# Autodesk Inventor assembly: AssemblyV1
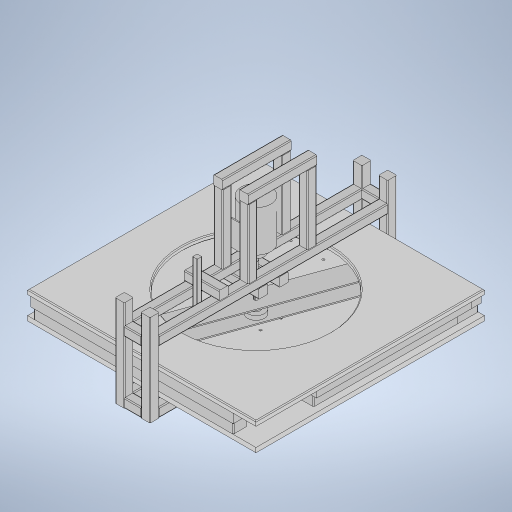
[picture p0: Inventor's stored thumbnail of the model, 512x512]
Saved by Autodesk Inventor 2024.4 (Build 284460000, 460)
## iProperties
Created: 2025-11-05
Part Number: AssemblyV1
Document SubType Name: Assembly
Designer: jonas
Author: jonas
## Documents named in this file (24)
- C:\Users\jonas\Documents\Studium\Master\3.Semester\StudentProject\SpinLauncher\drawingsV2\AssemblyV1.iam
- C:\Users\jonas\Documents\Studium\Master\3.Semester\StudentProject\SpinLauncher\drawingsV2\item40x40_1000.ipt
- C:\Users\jonas\Documents\Studium\Master\3.Semester\StudentProject\SpinLauncher\drawingsV2\item40x40_400.ipt
- C:\Users\jonas\Documents\Studium\Master\3.Semester\StudentProject\SpinLauncher\drawingsV2\item40x40_152_5.ipt
- C:\Users\jonas\Documents\Studium\Master\3.Semester\StudentProject\SpinLauncher\drawingsV2\FlanschKugellager15mm\7508860.iam
- C:\Users\jonas\Documents\Studium\Master\3.Semester\StudentProject\SpinLauncher\drawingsV2\motorOldV1.ipt
- C:\Users\jonas\Documents\Studium\Master\3.Semester\StudentProject\SpinLauncher\drawingsV2\item40x40_300.ipt
- C:\Users\jonas\Documents\Studium\Master\3.Semester\StudentProject\SpinLauncher\drawingsV2\ShaftNutV1.ipt
- C:\Users\jonas\Documents\Studium\Master\3.Semester\StudentProject\SpinLauncher\drawingsV2\rotorV1.ipt
- C:\Users\jonas\Documents\Studium\Master\3.Semester\StudentProject\SpinLauncher\drawingsV2\schaftManschetteV1.ipt
- C:\Users\jonas\Documents\Studium\Master\3.Semester\StudentProject\SpinLauncher\drawingsV2\item40x40_800.ipt
- C:\Users\jonas\Documents\Studium\Master\3.Semester\StudentProject\SpinLauncher\drawingsV2\item40x40_680.ipt
- C:\Users\jonas\Documents\Studium\Master\3.Semester\StudentProject\SpinLauncher\drawingsV2\item40x40_40.ipt
- C:\Users\jonas\Documents\Studium\Master\3.Semester\StudentProject\SpinLauncher\drawingsV2\boundaryWoodSchablone1V1.ipt
- C:\Users\jonas\Documents\Studium\Master\3.Semester\StudentProject\SpinLauncher\drawingsV2\boundaryWoodSchablone2V1.ipt
- C:\Users\jonas\Documents\Studium\Master\3.Semester\StudentProject\SpinLauncher\drawingsV2\boundaryWoodSchablone3V1.ipt
- C:\Users\jonas\Documents\Studium\Master\3.Semester\StudentProject\SpinLauncher\drawingsV2\groundPlateWoodV2.ipt
- C:\Users\jonas\Documents\Studium\Master\3.Semester\StudentProject\SpinLauncher\drawingsV2\item40x40_72_5.ipt
- C:\Users\jonas\Documents\Studium\Master\3.Semester\StudentProject\SpinLauncher\drawingsV2\FlanschV2.ipt
- C:\Users\jonas\Documents\Studium\Master\3.Semester\StudentProject\SpinLauncher\drawingsV2\AddBoundary1V1.ipt
- C:\Users\jonas\Documents\Studium\Master\3.Semester\StudentProject\SpinLauncher\drawingsV2\AddBoundary2V1.ipt
- C:\Users\jonas\Documents\Studium\Master\3.Semester\StudentProject\SpinLauncher\drawingsV2\topPlateWoodV1.ipt
- C:\Users\jonas\Documents\Studium\Master\3.Semester\StudentProject\SpinLauncher\drawingsV2\MagnetHolderV1.ipt
- C:\Users\jonas\Documents\Studium\Master\3.Semester\StudentProject\SpinLauncher\drawingsV2\MagnetShaft.ipt
## Components (55 placed, 23 different names)
1. item40x40_1000:1 — Mate:1, Mate:4, Flush:1, Flush:4, Flush:5, Flush:6, Flush:9, Flush:20, Flush:21, Flush:103, Mate:89, Mate:90
2. item40x40_1000:2 — Mate:2, Mate:3, Flush:2, Flush:3, Flush:7, Flush:8, Flush:9, Mate:11, Mate:12
3. item40x40_1000:3 — Flush:10, Mate:5, Flush:12, Mate:13, Mate:14, Flush:18, Flush:19, Mate:26, Flush:34, Mate:30, Flush:39, Mate:144, Flush:148
4. item40x40_1000:4 — Mate:6, Flush:11, Flush:12, Mate:25, Flush:33, Mate:29, Flush:40, Flush:129, Flush:133
5. item40x40_400:1 — Mate:2, Flush:2, Flush:3, Mate:6, Flush:11, Flush:13, Mate:92, Mate:125, Mate:126, Flush:130
6. item40x40_400:2 — Mate:1, Flush:1, Flush:4, Flush:10, Mate:5, Flush:13, Flush:127, Flush:128
7. item40x40_400:3 — Mate:3, Flush:7, Flush:8, Mate:127, Mate:128
8. item40x40_400:4 — Mate:4, Flush:5, Flush:6, Mate:91, Mate:113, Flush:131, Flush:132, Flush:134
9. item40x40_152_5:1 — Mate:13, Flush:18, Flush:23, Mate:22, Flush:45
10. item40x40_152_5:2 — Mate:12, Flush:21, Flush:22, Flush:46
11. item40x40_152_5:3 — Mate:14, Flush:19, Flush:22, Mate:15, Mate:23, Flush:46
12. item40x40_152_5:4 — Mate:11, Flush:20, Flush:23, Flush:45, Mate:38
13. 7508860:2 [sub-assembly] — Mate:15, Mate:20, Mate:22, Mate:23
14. motorOldV1:1 — Mate:20, Mate:31, Mate:32, Flush:43, Flush:44, Mate:33, Mate:34
15. item40x40_300:1 — Mate:26, Flush:34, Mate:28, Flush:37, Flush:38, Mate:31, Flush:44
16. item40x40_300:2 — Mate:25, Flush:33, Mate:27, Flush:35, Flush:36, Mate:32, Flush:43
17. item40x40_300:3 — Mate:27, Flush:35, Flush:36, Flush:42
18. item40x40_300:4 — Mate:28, Flush:37, Flush:38, Flush:41
19. item40x40_300:5 — Mate:29, Flush:40, Flush:42
20. item40x40_300:6 — Mate:30, Flush:39, Flush:41
21. ShaftNutV1:1 — Mate:33, Mate:34, Mate:36, Mate:39, Flush:103, Mate:82, Mate:83, Mate:105, Mate:110, Mate:114, Mate:123, Mate:130, Mate:133, Flush:136
22. rotorV1:1 — Mate:36, Mate:86, Mate:129, Flush:135, Mate:131, Mate:132
23. 7508860:3 [sub-assembly] — Mate:38, Mate:39
24. schaftManschetteV1:1 — Mate:82, Mate:86
25. schaftManschetteV1:2 — Mate:83, Mate:134
26. item40x40_800:1 — Mate:90, Mate:92, Flush:106, Mate:94, Mate:95, Mate:96, Flush:115, Flush:116, Flush:117, Flush:118
27. item40x40_800:2 — Mate:89, Mate:91, Flush:106, Flush:108, Flush:109, Mate:93, Mate:97, Mate:98, Flush:113, Flush:114, Flush:119, Flush:120
28. item40x40_680:1 — Flush:109, Mate:93
29. item40x40_680:2 — Flush:108, Mate:94, Mate:112
30. item40x40_40:1 — Mate:96, Flush:117, Flush:118
31. item40x40_40:2 — Mate:95, Flush:115, Flush:116
32. item40x40_40:3 — Mate:97, Flush:119, Flush:120
33. item40x40_40:4 — Mate:98, Flush:113, Flush:114
34. boundaryWoodSchablone1V1:1 — Mate:105, Mate:111, Mate:115, Flush:124, Mate:135, Flush:137, Flush:142, Mate:148, Flush:152
35. boundaryWoodSchablone3V1:1 — Mate:110, Mate:111, Mate:117
36. groundPlateWoodV2:1 — Mate:112, Mate:113, Mate:114, Mate:115, Mate:117, Flush:124, Mate:120, Mate:121, Mate:122, Flush:125, Mate:129, Flush:145, Flush:147, Mate:147
37. boundaryWoodSchablone1V1:2 — Mate:120, Flush:125, Flush:126, Mate:136, Flush:139, Flush:140
38. boundaryWoodSchablone2V1:2 — Mate:122, Mate:123, Mate:124, Flush:126, Mate:139
39. boundaryWoodSchablone3V1:2 — Mate:121, Mate:124
40. item40x40_72_5:1 — Mate:128, Flush:132, Flush:134
41. item40x40_72_5:2 — Mate:127, Flush:131, Flush:133
42. item40x40_72_5:3 — Mate:126, Flush:128, Flush:129
43. item40x40_72_5:4 — Mate:125, Flush:127, Flush:130
44. rotorV1:2 — Mate:130, Flush:135, Mate:131
45. FlanschV2:1 — Mate:132, Mate:133, Flush:136, Mate:134, Mate:142
46. AddBoundary1V1:1 — Mate:135, Flush:137, Mate:138, Flush:141, Flush:142, Flush:144, Flush:146
47. AddBoundary1V1:2 — Mate:136, Flush:139, Flush:140, Mate:140, Flush:143, Mate:141, Mate:143
48. AddBoundary2V1:1 — Mate:138, Flush:141
49. AddBoundary2V1:2 — Mate:139, Mate:140, Flush:143
50. topPlateWoodV1:1 — Mate:141, Flush:144, Flush:145
51. topPlateWoodV1:2 — Mate:143, Flush:146, Flush:147
52. item40x40_152_5:5 — Mate:144, Flush:148, Mate:146, Flush:151
53. MagnetHolderV1:1 — Flush:149, Flush:150, Mate:145
54. MagnetShaft:1 — Flush:149, Flush:150, Mate:145, Mate:146, Flush:151
55. boundaryWoodSchablone2V1:3 — Mate:147, Mate:148, Flush:152
## Relationships (151: Mate 78, Flush 73)
- Mate:1: item40x40_1000:1 ↔ item40x40_400:2
- Mate:2: item40x40_1000:2 ↔ item40x40_400:1
- Mate:3: item40x40_1000:2 ↔ item40x40_400:3
- Mate:4: item40x40_1000:1 ↔ item40x40_400:4
- Flush:1: item40x40_1000:1 ↔ item40x40_400:2
- Flush:2: item40x40_1000:2 ↔ item40x40_400:1
- Flush:3: item40x40_1000:2 ↔ item40x40_400:1
- Flush:4: item40x40_1000:1 ↔ item40x40_400:2
- Flush:5: item40x40_1000:1 ↔ item40x40_400:4
- Flush:6: item40x40_1000:1 ↔ item40x40_400:4
- Flush:7: item40x40_1000:2 ↔ item40x40_400:3
- Flush:8: item40x40_1000:2 ↔ item40x40_400:3
- Flush:9: item40x40_1000:1 ↔ item40x40_1000:2
- Flush:10: item40x40_1000:3 ↔ item40x40_400:2
- Mate:5: item40x40_1000:3 ↔ item40x40_400:2
- Mate:6: item40x40_1000:4 ↔ item40x40_400:1
- Flush:11: item40x40_1000:4 ↔ item40x40_400:1
- Flush:12: item40x40_1000:3 ↔ item40x40_1000:4
- Flush:13: item40x40_400:1 ↔ item40x40_400:2
- Mate:11: item40x40_1000:2 ↔ item40x40_152_5:4
- Mate:12: item40x40_1000:2 ↔ item40x40_152_5:2
- Mate:13: item40x40_1000:3 ↔ item40x40_152_5:1
- Mate:14: item40x40_1000:3 ↔ item40x40_152_5:3
- Flush:18: item40x40_1000:3 ↔ item40x40_152_5:1
- Flush:19: item40x40_1000:3 ↔ item40x40_152_5:3
- Flush:20: item40x40_1000:1 ↔ item40x40_152_5:4
- Flush:21: item40x40_1000:1 ↔ item40x40_152_5:2
- Flush:22: item40x40_152_5:2 ↔ item40x40_152_5:3
- Flush:23: item40x40_152_5:1 ↔ item40x40_152_5:4
- Mate:15: item40x40_152_5:3 ↔ 7508860:2
- Mate:20: 7508860:2 ↔ motorOldV1:1
- Mate:22 (-20 mm): item40x40_152_5:1 ↔ 7508860:2
- Mate:23 (-20 mm): item40x40_152_5:3 ↔ 7508860:2
- Mate:25: item40x40_1000:4 ↔ item40x40_300:2
- Flush:33: item40x40_1000:4 ↔ item40x40_300:2
- Mate:26: item40x40_1000:3 ↔ item40x40_300:1
- Flush:34: item40x40_1000:3 ↔ item40x40_300:1
- Mate:27: item40x40_300:2 ↔ item40x40_300:3
- Mate:28: item40x40_300:1 ↔ item40x40_300:4
- Flush:35: item40x40_300:2 ↔ item40x40_300:3
- Flush:36: item40x40_300:2 ↔ item40x40_300:3
- Flush:37: item40x40_300:1 ↔ item40x40_300:4
- Flush:38: item40x40_300:1 ↔ item40x40_300:4
- Mate:29: item40x40_1000:4 ↔ item40x40_300:5
- Mate:30: item40x40_1000:3 ↔ item40x40_300:6
- Flush:39: item40x40_1000:3 ↔ item40x40_300:6
- Flush:40: item40x40_1000:4 ↔ item40x40_300:5
- Flush:41: item40x40_300:4 ↔ item40x40_300:6
- Flush:42: item40x40_300:3 ↔ item40x40_300:5
- Mate:31: motorOldV1:1 ↔ item40x40_300:1
- Mate:32: motorOldV1:1 ↔ item40x40_300:2
- Flush:43 (8.75 mm): motorOldV1:1 ↔ item40x40_300:2
- Flush:44 (8.75 mm): motorOldV1:1 ↔ item40x40_300:1
- Flush:45: item40x40_152_5:1 ↔ item40x40_152_5:4
- Flush:46: item40x40_152_5:2 ↔ item40x40_152_5:3
- Mate:33: motorOldV1:1 ↔ ShaftNutV1:1
- Mate:34: motorOldV1:1 ↔ ShaftNutV1:1
- Mate:36: ShaftNutV1:1 ↔ rotorV1:1
- Mate:38: item40x40_152_5:4 ↔ 7508860:3
- Mate:39: ShaftNutV1:1 ↔ 7508860:3
- Flush:103 (10 mm): item40x40_1000:1 ↔ ShaftNutV1:1
- Mate:82: ShaftNutV1:1 ↔ schaftManschetteV1:1
- Mate:83: ShaftNutV1:1 ↔ schaftManschetteV1:2
- Mate:86: rotorV1:1 ↔ schaftManschetteV1:1
- Mate:89: item40x40_1000:1 ↔ item40x40_800:2
- Mate:90: item40x40_1000:1 ↔ item40x40_800:1
- Mate:91 (120 mm): item40x40_400:4 ↔ item40x40_800:2
- Mate:92 (120 mm): item40x40_400:1 ↔ item40x40_800:1
- Flush:106: item40x40_800:1 ↔ item40x40_800:2
- Flush:108: item40x40_800:2 ↔ item40x40_680:2
- Flush:109: item40x40_800:2 ↔ item40x40_680:1
- Mate:93: item40x40_800:2 ↔ item40x40_680:1
- Mate:94: item40x40_800:1 ↔ item40x40_680:2
- Mate:95: item40x40_800:1 ↔ item40x40_40:2
- Mate:96: item40x40_800:1 ↔ item40x40_40:1
- Mate:97: item40x40_800:2 ↔ item40x40_40:3
- Mate:98: item40x40_800:2 ↔ item40x40_40:4
- Flush:113: item40x40_800:2 ↔ item40x40_40:4
- Flush:114: item40x40_800:2 ↔ item40x40_40:4
- Flush:115: item40x40_800:1 ↔ item40x40_40:2
- Flush:116: item40x40_800:1 ↔ item40x40_40:2
- Flush:117: item40x40_800:1 ↔ item40x40_40:1
- Flush:118: item40x40_800:1 ↔ item40x40_40:1
- Flush:119: item40x40_800:2 ↔ item40x40_40:3
- Flush:120: item40x40_800:2 ↔ item40x40_40:3
- Mate:105: ShaftNutV1:1 ↔ boundaryWoodSchablone1V1:1
- Mate:110: ShaftNutV1:1 ↔ boundaryWoodSchablone3V1:1
- Mate:111: boundaryWoodSchablone1V1:1 ↔ boundaryWoodSchablone3V1:1
- Mate:112: item40x40_680:2 ↔ groundPlateWoodV2:1
- Mate:113: item40x40_400:4 ↔ groundPlateWoodV2:1
- Mate:114: ShaftNutV1:1 ↔ groundPlateWoodV2:1
- Mate:115: boundaryWoodSchablone1V1:1 ↔ groundPlateWoodV2:1
- Mate:117: boundaryWoodSchablone3V1:1 ↔ groundPlateWoodV2:1
- Flush:124: boundaryWoodSchablone1V1:1 ↔ groundPlateWoodV2:1
- [Mate]: boundaryWoodSchablone1V1:2 ↔ boundaryWoodSchablone2V1:2
- [Mate]: boundaryWoodSchablone1V1:2 ↔ boundaryWoodSchablone3V1:2
- Mate:120: groundPlateWoodV2:1 ↔ boundaryWoodSchablone1V1:2
- Mate:121: groundPlateWoodV2:1 ↔ boundaryWoodSchablone3V1:2
- Mate:122: groundPlateWoodV2:1 ↔ boundaryWoodSchablone2V1:2
- Mate:123: ShaftNutV1:1 ↔ boundaryWoodSchablone2V1:2
- Flush:125: groundPlateWoodV2:1 ↔ boundaryWoodSchablone1V1:2
- Mate:124: boundaryWoodSchablone2V1:2 ↔ boundaryWoodSchablone3V1:2
- Flush:126: boundaryWoodSchablone1V1:2 ↔ boundaryWoodSchablone2V1:2
- Mate:125: item40x40_400:1 ↔ item40x40_72_5:4
- Mate:126: item40x40_400:1 ↔ item40x40_72_5:3
- Mate:127: item40x40_400:3 ↔ item40x40_72_5:2
- Mate:128: item40x40_400:3 ↔ item40x40_72_5:1
- Flush:127: item40x40_400:2 ↔ item40x40_72_5:4
- Flush:128: item40x40_400:2 ↔ item40x40_72_5:3
- Flush:129: item40x40_1000:4 ↔ item40x40_72_5:3
- Flush:130: item40x40_400:1 ↔ item40x40_72_5:4
- Flush:131: item40x40_400:4 ↔ item40x40_72_5:2
- Flush:132: item40x40_400:4 ↔ item40x40_72_5:1
- Flush:133: item40x40_1000:4 ↔ item40x40_72_5:2
- Flush:134: item40x40_400:4 ↔ item40x40_72_5:1
- Mate:129 (3 mm): rotorV1:1 ↔ groundPlateWoodV2:1
- Mate:130: ShaftNutV1:1 ↔ rotorV1:2
- Flush:135: rotorV1:1 ↔ rotorV1:2
- Mate:131 (50 mm): rotorV1:1 ↔ rotorV1:2
- Mate:132: rotorV1:1 ↔ FlanschV2:1
- Mate:133: ShaftNutV1:1 ↔ FlanschV2:1
- Flush:136: ShaftNutV1:1 ↔ FlanschV2:1
- Mate:134: schaftManschetteV1:2 ↔ FlanschV2:1
- Mate:135: boundaryWoodSchablone1V1:1 ↔ AddBoundary1V1:1
- Flush:137: boundaryWoodSchablone1V1:1 ↔ AddBoundary1V1:1
- Mate:136: boundaryWoodSchablone1V1:2 ↔ AddBoundary1V1:2
- Flush:139: boundaryWoodSchablone1V1:2 ↔ AddBoundary1V1:2
- Flush:140: boundaryWoodSchablone1V1:2 ↔ AddBoundary1V1:2
- Mate:138: AddBoundary1V1:1 ↔ AddBoundary2V1:1
- Flush:141: AddBoundary1V1:1 ↔ AddBoundary2V1:1
- Flush:142: boundaryWoodSchablone1V1:1 ↔ AddBoundary1V1:1
- Mate:139: boundaryWoodSchablone2V1:2 ↔ AddBoundary2V1:2
- Mate:140: AddBoundary1V1:2 ↔ AddBoundary2V1:2
- Flush:143: AddBoundary1V1:2 ↔ AddBoundary2V1:2
- Mate:141: AddBoundary1V1:2 ↔ topPlateWoodV1:1
- Flush:144: AddBoundary1V1:1 ↔ topPlateWoodV1:1
- Flush:145: groundPlateWoodV2:1 ↔ topPlateWoodV1:1
- Mate:142: FlanschV2:1
- Mate:143: AddBoundary1V1:2 ↔ topPlateWoodV1:2
- Flush:146: AddBoundary1V1:1 ↔ topPlateWoodV1:2
- Flush:147: groundPlateWoodV2:1 ↔ topPlateWoodV1:2
- Mate:144: item40x40_1000:3 ↔ item40x40_152_5:5
- Flush:148: item40x40_1000:3 ↔ item40x40_152_5:5
- Flush:149: MagnetHolderV1:1 ↔ MagnetShaft:1
- Flush:150: MagnetHolderV1:1 ↔ MagnetShaft:1
- Mate:145: MagnetHolderV1:1 ↔ MagnetShaft:1
- Mate:146: item40x40_152_5:5 ↔ MagnetShaft:1
- Flush:151 (76.25 mm): item40x40_152_5:5 ↔ MagnetShaft:1
- Mate:147: groundPlateWoodV2:1 ↔ boundaryWoodSchablone2V1:3
- Mate:148: boundaryWoodSchablone1V1:1 ↔ boundaryWoodSchablone2V1:3
- Flush:152: boundaryWoodSchablone1V1:1 ↔ boundaryWoodSchablone2V1:3
## Named parameters: d280_d267 = 0 mm, d281_d272 = 0 mm
